# Autodesk Inventor assembly: Z
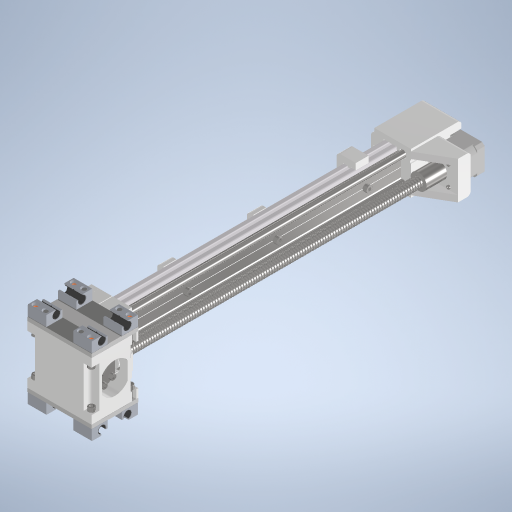
[picture p0: Inventor's stored thumbnail of the model, 512x512]
Saved by Autodesk Inventor 2024 (Build 280153000, 153)
## iProperties
Created: 2022-04-26
Part Number: Z
Document SubType Name: Assembly
Designer: mikoma
Author: mikoma
## Documents named in this file (30)
- D:\@home\mikoma\Dokumenty\DR\CartesianRobotsDigitalTwin\model\Workspaces\Obszar roboczy\assembly_v3\Z\Z.iam
- D:\@home\mikoma\Dokumenty\DR\CartesianRobotsDigitalTwin\model\Workspaces\Obszar roboczy\content\igus\WW_10_40_10_2.ipt
- D:\@home\mikoma\Dokumenty\DR\CartesianRobotsDigitalTwin\model\Workspaces\Obszar roboczy\assembly_v3\Z\ZCarriage.ipt
- D:\@home\mikoma\Dokumenty\DR\CartesianRobotsDigitalTwin\model\Workspaces\Obszar roboczy\content\manipulatorSharedParts\Cartesian1_BallNut.ipt
- D:\@home\mikoma\Dokumenty\DR\CartesianRobotsDigitalTwin\model\Workspaces\Obszar roboczy\content\manipulatorSharedParts\Cartesian2_BallBearing_25x37x7.ipt
- D:\@home\mikoma\Dokumenty\DR\CartesianRobotsDigitalTwin\model\Workspaces\Obszar roboczy\CC\pl-PL\ISO 4762(1)\DIN EN ISO 4762 - M6 x 30.ipt
- D:\@home\mikoma\Dokumenty\DR\CartesianRobotsDigitalTwin\model\Workspaces\Obszar roboczy\assembly_v3\Z\ZCarriageBackHolder.ipt
- D:\@home\mikoma\Dokumenty\DR\CartesianRobotsDigitalTwin\model\Workspaces\Obszar roboczy\assembly_v3\Z\ZCarriageFrontHolder.ipt
- D:\@home\mikoma\Dokumenty\DR\CartesianRobotsDigitalTwin\model\Workspaces\Obszar roboczy\assembly_v3\Z\ZScrewEndCup.ipt
- D:\@home\mikoma\Dokumenty\DR\CartesianRobotsDigitalTwin\model\Workspaces\Obszar roboczy\assembly_v3\Z\WS_10_40_Z.ipt
- D:\@home\mikoma\Dokumenty\DR\CartesianRobotsDigitalTwin\model\Workspaces\Obszar roboczy\content\item\item_0037003_Profile_5_20x20_L=564_1.ipt
- D:\@home\mikoma\Dokumenty\DR\CartesianRobotsDigitalTwin\model\Workspaces\Obszar roboczy\assembly_v3\Z\ZTop.ipt
- D:\@home\mikoma\Dokumenty\DR\CartesianRobotsDigitalTwin\model\Workspaces\Obszar roboczy\content\manipulatorSharedParts\Cartesian1_12_12_Clutch.ipt
- D:\@home\mikoma\Dokumenty\DR\CartesianRobotsDigitalTwin\model\Workspaces\Obszar roboczy\content\manipulatorSharedParts\Cartesian1_TrapezoidalScrew.ipt
- D:\@home\mikoma\Dokumenty\DR\CartesianRobotsDigitalTwin\model\Workspaces\Obszar roboczy\assembly_v3\Z\ZItemMount.ipt
- D:\@home\mikoma\Dokumenty\DR\CartesianRobotsDigitalTwin\model\Workspaces\Obszar roboczy\content\manipulatorSharedParts\stopSw.ipt
- D:\@home\mikoma\Dokumenty\DR\CartesianRobotsDigitalTwin\model\Workspaces\Obszar roboczy\content\manipulatorSharedParts\Connector_female.ipt
- D:\@home\mikoma\Dokumenty\DR\CartesianRobotsDigitalTwin\model\Workspaces\Obszar roboczy\CC\pl-PL\ISO 4762(1)\DIN EN ISO 4762 - M5 x 40.ipt
- D:\@home\mikoma\Dokumenty\DR\CartesianRobotsDigitalTwin\model\Workspaces\Obszar roboczy\CC\pl-PL\ISO 4032(2)\ISO 4032 - M5 - ISO.ipt
- D:\@home\mikoma\Dokumenty\DR\CartesianRobotsDigitalTwin\model\Workspaces\Obszar roboczy\assembly_v3\Z\ZItemMountCable.ipt
- D:\@home\mikoma\Dokumenty\DR\CartesianRobotsDigitalTwin\model\Workspaces\Obszar roboczy\assembly_v3\Z\ZTopCable.ipt
- D:\@home\mikoma\Dokumenty\DR\CartesianRobotsDigitalTwin\model\Workspaces\Obszar roboczy\CC\pl-PL\ISO 4762(2)\ISO 4762 - M4 x 25ISO.ipt
- D:\@home\mikoma\Dokumenty\DR\CartesianRobotsDigitalTwin\model\Workspaces\Obszar roboczy\CC\pl-PL\ISO 4762(1)\DIN EN ISO 4762 - M6 x 25.ipt
- D:\@home\mikoma\Dokumenty\DR\CartesianRobotsDigitalTwin\model\Workspaces\Obszar roboczy\CC\pl-PL\ISO 4762(1)\DIN EN ISO 4762 - M6 x 55.ipt
- D:\@home\mikoma\Dokumenty\DR\CartesianRobotsDigitalTwin\model\Workspaces\Obszar roboczy\CC\pl-PL\ISO 4032(2)\ISO 4032 - M6 - ISO.ipt
- D:\@home\mikoma\Dokumenty\DR\CartesianRobotsDigitalTwin\model\Workspaces\Obszar roboczy\CC\pl-PL\DIN 7984\DIN 7984 - M4 x 14.ipt
- D:\@home\mikoma\Dokumenty\DR\CartesianRobotsDigitalTwin\model\Workspaces\Obszar roboczy\CC\pl-PL\ISO 4762(1)\DIN EN ISO 4762 - M6 x 35.ipt
- D:\@home\mikoma\Dokumenty\DR\CartesianRobotsDigitalTwin\model\Workspaces\Obszar roboczy\CC\pl-PL\DIN 7984\DIN 7984 - M3 x 14.ipt
- D:\@home\mikoma\Dokumenty\DR\CartesianRobotsDigitalTwin\model\Workspaces\Obszar roboczy\content\item\item_0037006_Wpust_przesuwny_5_St_M4_1.ipt
- D:\@home\mikoma\Dokumenty\DR\CartesianRobotsDigitalTwin\model\Workspaces\Obszar roboczy\content\nema17\17HS4401\17HS4401.ipt
## Components (75 placed, 29 different names)
1. WW_10_40_10_2:1 — Zestawiające:14, Zestawiające:15, Zestawiające:18, Zestawiające:19
2. WW_10_40_10_2:2 — Zestawiające:16, Zestawiające:17, Zestawiające:18
3. ZCarriage:1 — Równoległe:2, Zestawiające:13, Równoległe:3, Zestawiające:14, Zestawiające:15, Zestawiające:16, Zestawiające:17, Zestawiające:20, Kątowe:1, Zestawiające:21, Zestawiające:22, Zestawiające:23, Zestawiające:24, Zestawiające:25, Zestawiające:26, Zestawiające:27, Zestawiające:28, Równoległe:4, Równoległe:5, Równoległe:6, Zestawiające:29, Zestawiające:30, Zestawiające:31, Zestawiające:34, Zestawiające:35, Zestawiające:36, Zestawiające:39, Zestawiające:40, Zestawiające:56, Zestawiające:57, Zestawiające:58, Kątowe:3, Zestawiające:62, Zestawiające:80, Zestawiające:81, Zestawiające:82, Zestawiające:83, Zestawiające:84, Zestawiające:85, Zestawiające:86, Zestawiające:87, Zestawiające:88, Zestawiające:89, Zestawiające:90, Zestawiające:91, Kątowe:4, Zestawiające:101, Kątowe:5, Zestawiające:103, Kątowe:6, Zestawiające:105, Kątowe:7, Zestawiające:107, Kątowe:8, Zestawiające:109
4. Cartesian1_BallNut:1 — Zestawiające:20, Kątowe:1, Zestawiające:21, Zestawiające:59, Zestawiające:60, Zestawiające:70, Zestawiające:71, Zestawiające:72, Zestawiające:73, Zestawiające:74, Zestawiające:75, Zestawiające:76, Zestawiające:77, Zestawiające:78, Zestawiające:79
5. Cartesian2_BallBearing_25x37x7:1 — Zestawiające:22, Zestawiające:23
6. ZCarriageBackHolder:1 — Zestawiające:28, Równoległe:4, Równoległe:5, Kątowe:9, Zestawiające:111, Kątowe:10, Zestawiające:113, Kątowe:11, Zestawiające:116, Kątowe:12, Zestawiające:118, Zestawiające:125
7. ZScrewEndCup:1 — Zestawiające:46
8. ZCarriageFrontHolder:1 — Równoległe:6, Zestawiające:29, Zestawiające:30, Zestawiające:31, Zestawiające:32, Zestawiające:33, Równoległe:7, Zestawiające:54, Zestawiające:55, Zestawiające:92, Zestawiające:93, Zestawiające:94, Zestawiające:95, Zestawiające:96, Zestawiające:97, Zestawiające:98, Zestawiające:99
9. WS_10_40_Z:1 — Zestawiające:32, Zestawiające:33, Zestawiające:34, Zestawiające:37, Zestawiające:38, Zestawiające:41, Zestawiające:42, Zestawiające:141, Zestawiające:143, Zestawiające:145
10. item_0037003_Profile_5_20x20_L=564_1:1 — Zestawiające:38, Zestawiające:39, Zestawiające:40, Zestawiające:50, Zestawiające:159, Zestawiające:161, Zestawiające:165, Zestawiające:169
11. item_0037003_Profile_5_20x20_L=564_1:2 — Zestawiające:35, Zestawiające:36, Zestawiające:37, Zestawiające:43, Zestawiające:51, Zestawiające:52, Zestawiające:53, Zestawiające:63, Zestawiające:64, Zestawiające:157, Zestawiające:163, Zestawiające:167, Zestawiające:171
12. ZTop:1 — Zestawiające:41, Zestawiające:42, Zestawiające:43, Zestawiające:49, Zestawiające:65, Zestawiające:66, Zestawiające:67, Zestawiające:148, Zestawiające:149, Zestawiające:150, Zestawiające:151, Zestawiające:152, Zestawiające:153, Zestawiające:154, Zestawiające:155, Mate:174
13. Cartesian1_12_12_Clutch:1 — Zestawiające:47, Zestawiające:48, Zestawiające:49
14. Cartesian1_TrapezoidalScrew:1 — Zestawiające:46, Zestawiające:47, Zestawiające:48
15. ZItemMount:1 — Zestawiające:50, Zestawiające:51, Zestawiające:119, Kątowe:13, Zestawiające:120, Zestawiające:125, Zestawiające:126, Zestawiające:136, Zestawiające:137, Zestawiające:138, Zestawiające:139, Kątowe:16, Kątowe:17
16. ZItemMount:2 — Zestawiające:52, Zestawiające:53, Zestawiające:121, Kątowe:14, Zestawiające:122, Zestawiające:126, Zestawiające:127, Zestawiające:132, Zestawiające:133, Zestawiające:134, Zestawiające:135, Kątowe:18, Kątowe:19
17. stopSw:1 — Równoległe:7, Zestawiające:54, Zestawiające:55
18. Connector_female:1 — Zestawiające:56, Zestawiające:57, Zestawiające:58
19. ZItemMountCable:1 — Zestawiające:63, Zestawiające:64, Zestawiające:123, Kątowe:15, Zestawiające:124, Zestawiające:127, Zestawiające:128, Zestawiające:129, Zestawiające:130, Zestawiające:131, Kątowe:20, Kątowe:21
20. ZTopCable:1 — Zestawiające:65, Zestawiające:66, Zestawiające:67, Zestawiające:146, Zestawiające:147, Kątowe:22, Kątowe:23, Zestawiające:172, Zestawiające:173
21. 17HS4401:1 — Mate:174, Mate:175, Mate:176
22. DIN EN ISO 4762 M6 x 30:2 — Zestawiające:26, Zestawiające:27
23. DIN EN ISO 4762 M6 x 25:1 — Zestawiające:24, Zestawiające:25
24. ISO 4032 M5:1 — Zestawiające:61, Kątowe:3, Zestawiające:62
25. DIN EN ISO 4762 M5 x 40:1 — Zestawiające:59, Zestawiające:60, Zestawiające:61
26. DIN EN ISO 4762 M6 x 30:8 — Zestawiające:90, Zestawiające:91
27. DIN EN ISO 4762 M6 x 30:7 — Zestawiające:88, Zestawiające:89
28. DIN EN ISO 4762 M6 x 30:6 — Zestawiające:86, Zestawiające:87
29. DIN EN ISO 4762 M6 x 30:5 — Zestawiające:84, Zestawiające:85
30. DIN EN ISO 4762 M6 x 30:4 — Zestawiające:82, Zestawiające:83
31. DIN EN ISO 4762 M6 x 25:2 — Zestawiające:80, Zestawiające:81
32. DIN EN ISO 4762 M5 x 40:6 — Zestawiające:74, Zestawiające:77, Zestawiające:104
33. DIN EN ISO 4762 M5 x 40:5 — Zestawiające:73, Zestawiające:78, Zestawiające:106
34. DIN EN ISO 4762 M5 x 40:4 — Zestawiające:72, Zestawiające:79, Zestawiające:108
35. DIN EN ISO 4762 M5 x 40:3 — Zestawiające:71, Zestawiające:75, Zestawiające:102
36. DIN EN ISO 4762 M5 x 40:2 — Zestawiające:70, Zestawiające:76, Zestawiające:100
37. DIN 7984 M3 x 14:4 — Zestawiające:154, Zestawiające:155
38. DIN 7984 M3 x 14:3 — Zestawiające:152, Zestawiające:153, Mate:175
39. DIN 7984 M3 x 14:2 — Zestawiające:150, Zestawiające:151
40. DIN 7984 M3 x 14:1 — Zestawiające:148, Zestawiające:149, Mate:176
41. ISO 4762 M4 x 25:2 — Zestawiające:146, Zestawiające:147, Zestawiające:170
42. DIN EN ISO 4762 M6 x 35:3 — Zestawiające:144, Zestawiające:145
43. DIN EN ISO 4762 M6 x 35:2 — Zestawiające:142, Zestawiające:143
44. DIN EN ISO 4762 M6 x 35:1 — Zestawiające:140, Zestawiające:141
45. DIN 7984 M4 x 14:6 — Zestawiające:138, Zestawiające:139, Zestawiające:156
46. DIN 7984 M4 x 14:5 — Zestawiające:136, Zestawiające:137, Zestawiające:158
47. DIN 7984 M4 x 14:4 — Zestawiające:134, Zestawiające:135, Zestawiające:162
48. DIN 7984 M4 x 14:3 — Zestawiające:132, Zestawiające:133, Zestawiające:160
49. DIN 7984 M4 x 14:2 — Zestawiające:130, Zestawiające:131, Zestawiające:166
50. DIN 7984 M4 x 14:1 — Zestawiające:128, Zestawiające:129, Zestawiające:164
51. ISO 4032 M6:7 — Zestawiające:123, Kątowe:15, Zestawiające:124, Zestawiające:144
52. ISO 4032 M6:6 — Zestawiające:121, Kątowe:14, Zestawiające:122, Zestawiające:142
53. ISO 4032 M6:5 — Zestawiające:119, Kątowe:13, Zestawiające:120, Zestawiające:140
54. ISO 4032 M6:4 — Zestawiające:117, Kątowe:12, Zestawiające:118
55. ISO 4032 M6:3 — Zestawiające:114, Zestawiające:115, Kątowe:11, Zestawiające:116
56. ISO 4032 M6:2 — Zestawiające:112, Kątowe:10, Zestawiające:113
57. ISO 4032 M6:1 — Zestawiające:110, Kątowe:9, Zestawiające:111
58. ISO 4032 M5:6 — Kątowe:8, Zestawiające:108, Zestawiające:109
59. ISO 4032 M5:5 — Kątowe:7, Zestawiające:106, Zestawiające:107
60. ISO 4032 M5:4 — Kątowe:6, Zestawiające:104, Zestawiające:105
61. ISO 4032 M5:3 — Kątowe:5, Zestawiające:102, Zestawiające:103
62. ISO 4032 M5:2 — Zestawiające:100, Kątowe:4, Zestawiające:101
63. DIN EN ISO 4762 M6 x 55:4 — Zestawiające:98, Zestawiające:99, Zestawiające:110
64. DIN EN ISO 4762 M6 x 55:3 — Zestawiające:96, Zestawiające:97, Zestawiające:112
65. DIN EN ISO 4762 M6 x 55:2 — Zestawiające:94, Zestawiające:95, Zestawiające:117
66. DIN EN ISO 4762 M6 x 55:1 — Zestawiające:92, Zestawiające:93, Zestawiające:114, Zestawiające:115
67. item_0037006_Wpust_przesuwny_5_St_M4_1:1 — Zestawiające:156, Kątowe:16, Zestawiające:157
68. item_0037006_Wpust_przesuwny_5_St_M4_1:2 — Zestawiające:158, Kątowe:17, Zestawiające:159
69. item_0037006_Wpust_przesuwny_5_St_M4_1:3 — Zestawiające:160, Kątowe:18, Zestawiające:161
70. item_0037006_Wpust_przesuwny_5_St_M4_1:4 — Zestawiające:162, Kątowe:19, Zestawiające:163
71. item_0037006_Wpust_przesuwny_5_St_M4_1:5 — Zestawiające:164, Kątowe:20, Zestawiające:165
72. item_0037006_Wpust_przesuwny_5_St_M4_1:6 — Zestawiające:166, Kątowe:21, Zestawiające:167
73. item_0037006_Wpust_przesuwny_5_St_M4_1:7 — Kątowe:22, Zestawiające:169
74. item_0037006_Wpust_przesuwny_5_St_M4_1:8 — Zestawiające:170, Kątowe:23, Zestawiające:171
75. ISO 4762 M4 x 25:3 — Zestawiające:172, Zestawiające:173
## Relationships (189: Mate 161, Angle 22, Flush 6)
- [Mate]: Cartesian2_BallBearing_25x37x7:1 ↔ ZScrewEndCup:1
- [Mate]: Cartesian2_BallBearing_25x37x7:1 ↔ ZScrewEndCup:1
- Równoległe:2 [Flush]: ZCarriage:1
- Zestawiające:13 [Mate]: ZCarriage:1
- Równoległe:3 [Flush]: ZCarriage:1
- Zestawiające:14 [Mate]: WW_10_40_10_2:1 ↔ ZCarriage:1
- Zestawiające:15 [Mate]: WW_10_40_10_2:1 ↔ ZCarriage:1
- Zestawiające:16 [Mate]: WW_10_40_10_2:2 ↔ ZCarriage:1
- Zestawiające:17 [Mate]: WW_10_40_10_2:2 ↔ ZCarriage:1
- Zestawiające:18 [Mate] (120 mm): WW_10_40_10_2:1 ↔ WW_10_40_10_2:2
- Zestawiające:19 [Mate] (-67.5 mm): WW_10_40_10_2:1
- Zestawiające:20 [Mate]: ZCarriage:1 ↔ Cartesian1_BallNut:1
- Kątowe:1 [Angle] (0 deg): ZCarriage:1 ↔ Cartesian1_BallNut:1
- Zestawiające:21 [Mate]: ZCarriage:1 ↔ Cartesian1_BallNut:1
- Zestawiające:22 [Mate]: ZCarriage:1 ↔ Cartesian2_BallBearing_25x37x7:1
- Zestawiające:23 [Mate]: ZCarriage:1 ↔ Cartesian2_BallBearing_25x37x7:1
- Zestawiające:24 [Mate]: ZCarriage:1 ↔ DIN EN ISO 4762 M6 x 25:1
- Zestawiające:25 [Mate]: ZCarriage:1 ↔ DIN EN ISO 4762 M6 x 25:1
- Zestawiające:26 [Mate]: ZCarriage:1 ↔ DIN EN ISO 4762 M6 x 30:2
- Zestawiające:27 [Mate]: ZCarriage:1 ↔ DIN EN ISO 4762 M6 x 30:2
- Zestawiające:28 [Mate]: ZCarriage:1 ↔ ZCarriageBackHolder:1
- Równoległe:4 [Flush]: ZCarriage:1 ↔ ZCarriageBackHolder:1
- Równoległe:5 [Flush]: ZCarriage:1 ↔ ZCarriageBackHolder:1
- Równoległe:6 [Flush]: ZCarriage:1 ↔ ZCarriageFrontHolder:1
- Zestawiające:29 [Mate]: ZCarriage:1 ↔ ZCarriageFrontHolder:1
- Zestawiające:30 [Mate]: ZCarriage:1 ↔ ZCarriageFrontHolder:1
- Zestawiające:31 [Mate]: ZCarriage:1 ↔ ZCarriageFrontHolder:1
- Zestawiające:32 [Mate]: ZCarriageFrontHolder:1 ↔ WS_10_40_Z:1
- Zestawiające:33 [Mate]: ZCarriageFrontHolder:1 ↔ WS_10_40_Z:1
- Zestawiające:34 [Mate]: ZCarriage:1 ↔ WS_10_40_Z:1
- Zestawiające:35 [Mate]: ZCarriage:1 ↔ item_0037003_Profile_5_20x20_L=564_1:2
- Zestawiające:36 [Mate]: ZCarriage:1 ↔ item_0037003_Profile_5_20x20_L=564_1:2
- Zestawiające:37 [Mate]: WS_10_40_Z:1 ↔ item_0037003_Profile_5_20x20_L=564_1:2
- Zestawiające:38 [Mate]: WS_10_40_Z:1 ↔ item_0037003_Profile_5_20x20_L=564_1:1
- Zestawiające:39 [Mate]: ZCarriage:1 ↔ item_0037003_Profile_5_20x20_L=564_1:1
- Zestawiające:40 [Mate]: ZCarriage:1 ↔ item_0037003_Profile_5_20x20_L=564_1:1
- Zestawiające:41 [Mate]: WS_10_40_Z:1 ↔ ZTop:1
- Zestawiające:42 [Mate]: WS_10_40_Z:1 ↔ ZTop:1
- Zestawiające:43 [Mate]: item_0037003_Profile_5_20x20_L=564_1:2 ↔ ZTop:1
- Zestawiające:46 [Mate]: ZScrewEndCup:1 ↔ Cartesian1_TrapezoidalScrew:1
- Zestawiające:47 [Mate]: Cartesian1_12_12_Clutch:1 ↔ Cartesian1_TrapezoidalScrew:1
- Zestawiające:48 [Mate]: Cartesian1_12_12_Clutch:1 ↔ Cartesian1_TrapezoidalScrew:1
- Zestawiające:49 [Mate]: ZTop:1 ↔ Cartesian1_12_12_Clutch:1
- Zestawiające:50 [Mate]: item_0037003_Profile_5_20x20_L=564_1:1 ↔ ZItemMount:1
- Zestawiające:51 [Mate]: item_0037003_Profile_5_20x20_L=564_1:2 ↔ ZItemMount:1
- Zestawiające:52 [Mate]: item_0037003_Profile_5_20x20_L=564_1:2 ↔ ZItemMount:2
- Zestawiające:53 [Mate]: item_0037003_Profile_5_20x20_L=564_1:2 ↔ ZItemMount:2
- Równoległe:7 [Flush] (-1 mm): ZCarriageFrontHolder:1 ↔ stopSw:1
- Zestawiające:54 [Mate]: ZCarriageFrontHolder:1 ↔ stopSw:1
- Zestawiające:55 [Mate]: ZCarriageFrontHolder:1 ↔ stopSw:1
- Zestawiające:56 [Mate]: ZCarriage:1 ↔ Connector_female:1
- Zestawiające:57 [Mate]: ZCarriage:1 ↔ Connector_female:1
- Zestawiające:58 [Mate]: ZCarriage:1 ↔ Connector_female:1
- Zestawiające:59 [Mate]: Cartesian1_BallNut:1 ↔ DIN EN ISO 4762 M5 x 40:1
- Zestawiające:60 [Mate]: Cartesian1_BallNut:1 ↔ DIN EN ISO 4762 M5 x 40:1
- Zestawiające:61 [Mate]: ISO 4032 M5:1 ↔ DIN EN ISO 4762 M5 x 40:1
- Kątowe:3 [Angle] (0 deg): ZCarriage:1 ↔ ISO 4032 M5:1
- Zestawiające:62 [Mate]: ZCarriage:1 ↔ ISO 4032 M5:1
- Zestawiające:63 [Mate]: item_0037003_Profile_5_20x20_L=564_1:2 ↔ ZItemMountCable:1
- Zestawiające:64 [Mate]: item_0037003_Profile_5_20x20_L=564_1:2 ↔ ZItemMountCable:1
- Zestawiające:65 [Mate]: ZTop:1 ↔ ZTopCable:1
- Zestawiające:66 [Mate]: ZTop:1 ↔ ZTopCable:1
- Zestawiające:67 [Mate]: ZTop:1 ↔ ZTopCable:1
- Zestawiające:70 [Mate]: Cartesian1_BallNut:1 ↔ DIN EN ISO 4762 M5 x 40:2
- Zestawiające:71 [Mate]: Cartesian1_BallNut:1 ↔ DIN EN ISO 4762 M5 x 40:3
- Zestawiające:72 [Mate]: Cartesian1_BallNut:1 ↔ DIN EN ISO 4762 M5 x 40:4
- Zestawiające:73 [Mate]: Cartesian1_BallNut:1 ↔ DIN EN ISO 4762 M5 x 40:5
- Zestawiające:74 [Mate]: Cartesian1_BallNut:1 ↔ DIN EN ISO 4762 M5 x 40:6
- Zestawiające:75 [Mate]: Cartesian1_BallNut:1 ↔ DIN EN ISO 4762 M5 x 40:3
- Zestawiające:76 [Mate]: Cartesian1_BallNut:1 ↔ DIN EN ISO 4762 M5 x 40:2
- Zestawiające:77 [Mate]: Cartesian1_BallNut:1 ↔ DIN EN ISO 4762 M5 x 40:6
- Zestawiające:78 [Mate]: Cartesian1_BallNut:1 ↔ DIN EN ISO 4762 M5 x 40:5
- Zestawiające:79 [Mate]: Cartesian1_BallNut:1 ↔ DIN EN ISO 4762 M5 x 40:4
- Zestawiające:80 [Mate]: ZCarriage:1 ↔ DIN EN ISO 4762 M6 x 25:2
- Zestawiające:81 [Mate]: ZCarriage:1 ↔ DIN EN ISO 4762 M6 x 25:2
- Zestawiające:82 [Mate]: ZCarriage:1 ↔ DIN EN ISO 4762 M6 x 30:4
- Zestawiające:83 [Mate]: ZCarriage:1 ↔ DIN EN ISO 4762 M6 x 30:4
- Zestawiające:84 [Mate]: ZCarriage:1 ↔ DIN EN ISO 4762 M6 x 30:5
- Zestawiające:85 [Mate]: ZCarriage:1 ↔ DIN EN ISO 4762 M6 x 30:5
- Zestawiające:86 [Mate]: ZCarriage:1 ↔ DIN EN ISO 4762 M6 x 30:6
- Zestawiające:87 [Mate]: ZCarriage:1 ↔ DIN EN ISO 4762 M6 x 30:6
- Zestawiające:88 [Mate]: ZCarriage:1 ↔ DIN EN ISO 4762 M6 x 30:7
- Zestawiające:89 [Mate]: ZCarriage:1 ↔ DIN EN ISO 4762 M6 x 30:7
- Zestawiające:90 [Mate]: ZCarriage:1 ↔ DIN EN ISO 4762 M6 x 30:8
- Zestawiające:91 [Mate]: ZCarriage:1 ↔ DIN EN ISO 4762 M6 x 30:8
- Zestawiające:92 [Mate]: ZCarriageFrontHolder:1 ↔ DIN EN ISO 4762 M6 x 55:1
- Zestawiające:93 [Mate]: ZCarriageFrontHolder:1 ↔ DIN EN ISO 4762 M6 x 55:1
- Zestawiające:94 [Mate]: ZCarriageFrontHolder:1 ↔ DIN EN ISO 4762 M6 x 55:2
- Zestawiające:95 [Mate]: ZCarriageFrontHolder:1 ↔ DIN EN ISO 4762 M6 x 55:2
- Zestawiające:96 [Mate]: ZCarriageFrontHolder:1 ↔ DIN EN ISO 4762 M6 x 55:3
- Zestawiające:97 [Mate]: ZCarriageFrontHolder:1 ↔ DIN EN ISO 4762 M6 x 55:3
- Zestawiające:98 [Mate]: ZCarriageFrontHolder:1 ↔ DIN EN ISO 4762 M6 x 55:4
- Zestawiające:99 [Mate]: ZCarriageFrontHolder:1 ↔ DIN EN ISO 4762 M6 x 55:4
- Zestawiające:100 [Mate]: DIN EN ISO 4762 M5 x 40:2 ↔ ISO 4032 M5:2
- Kątowe:4 [Angle] (0 deg): ZCarriage:1 ↔ ISO 4032 M5:2
- Zestawiające:101 [Mate]: ZCarriage:1 ↔ ISO 4032 M5:2
- Kątowe:5 [Angle] (0 deg): ZCarriage:1 ↔ ISO 4032 M5:3
- Zestawiające:102 [Mate]: DIN EN ISO 4762 M5 x 40:3 ↔ ISO 4032 M5:3
- Zestawiające:103 [Mate]: ZCarriage:1 ↔ ISO 4032 M5:3
- Kątowe:6 [Angle] (0 deg): ZCarriage:1 ↔ ISO 4032 M5:4
- Zestawiające:104 [Mate]: DIN EN ISO 4762 M5 x 40:6 ↔ ISO 4032 M5:4
- Zestawiające:105 [Mate]: ZCarriage:1 ↔ ISO 4032 M5:4
- Kątowe:7 [Angle] (0 deg): ZCarriage:1 ↔ ISO 4032 M5:5
- Zestawiające:106 [Mate]: DIN EN ISO 4762 M5 x 40:5 ↔ ISO 4032 M5:5
- Zestawiające:107 [Mate]: ZCarriage:1 ↔ ISO 4032 M5:5
- Kątowe:8 [Angle] (0 deg): ZCarriage:1 ↔ ISO 4032 M5:6
- Zestawiające:108 [Mate]: DIN EN ISO 4762 M5 x 40:4 ↔ ISO 4032 M5:6
- Zestawiające:109 [Mate]: ZCarriage:1 ↔ ISO 4032 M5:6
- Zestawiające:110 [Mate]: ISO 4032 M6:1 ↔ DIN EN ISO 4762 M6 x 55:4
- Kątowe:9 [Angle] (0 deg): ZCarriageBackHolder:1 ↔ ISO 4032 M6:1
- Zestawiające:111 [Mate]: ZCarriageBackHolder:1 ↔ ISO 4032 M6:1
- Zestawiające:112 [Mate]: ISO 4032 M6:2 ↔ DIN EN ISO 4762 M6 x 55:3
- Kątowe:10 [Angle] (0 deg): ZCarriageBackHolder:1 ↔ ISO 4032 M6:2
- Zestawiające:113 [Mate]: ZCarriageBackHolder:1 ↔ ISO 4032 M6:2
- Zestawiające:114 [Mate]: ISO 4032 M6:3 ↔ DIN EN ISO 4762 M6 x 55:1
- Zestawiające:115 [Mate]: ISO 4032 M6:3 ↔ DIN EN ISO 4762 M6 x 55:1
- Kątowe:11 [Angle] (0 deg): ZCarriageBackHolder:1 ↔ ISO 4032 M6:3
- Zestawiające:116 [Mate]: ZCarriageBackHolder:1 ↔ ISO 4032 M6:3
- Zestawiające:117 [Mate]: ISO 4032 M6:4 ↔ DIN EN ISO 4762 M6 x 55:2
- Kątowe:12 [Angle] (0 deg): ZCarriageBackHolder:1 ↔ ISO 4032 M6:4
- Zestawiające:118 [Mate]: ZCarriageBackHolder:1 ↔ ISO 4032 M6:4
- Zestawiające:119 [Mate]: ZItemMount:1 ↔ ISO 4032 M6:5
- Kątowe:13 [Angle] (0 deg): ZItemMount:1 ↔ ISO 4032 M6:5
- Zestawiające:120 [Mate]: ZItemMount:1 ↔ ISO 4032 M6:5
- Zestawiające:121 [Mate]: ZItemMount:2 ↔ ISO 4032 M6:6
- Kątowe:14 [Angle] (0 deg): ZItemMount:2 ↔ ISO 4032 M6:6
- Zestawiające:122 [Mate]: ZItemMount:2 ↔ ISO 4032 M6:6
- Zestawiające:123 [Mate]: ZItemMountCable:1 ↔ ISO 4032 M6:7
- Kątowe:15 [Angle] (0 deg): ZItemMountCable:1 ↔ ISO 4032 M6:7
- Zestawiające:124 [Mate]: ZItemMountCable:1 ↔ ISO 4032 M6:7
- Zestawiające:125 [Mate] (100 mm): ZCarriageBackHolder:1 ↔ ZItemMount:1
- Zestawiające:126 [Mate] (120 mm): ZItemMount:1 ↔ ZItemMount:2
- Zestawiające:127 [Mate] (120 mm): ZItemMount:2 ↔ ZItemMountCable:1
- Zestawiające:128 [Mate]: ZItemMountCable:1 ↔ DIN 7984 M4 x 14:1
- Zestawiające:129 [Mate]: ZItemMountCable:1 ↔ DIN 7984 M4 x 14:1
- Zestawiające:130 [Mate]: ZItemMountCable:1 ↔ DIN 7984 M4 x 14:2
- Zestawiające:131 [Mate]: ZItemMountCable:1 ↔ DIN 7984 M4 x 14:2
- Zestawiające:132 [Mate]: ZItemMount:2 ↔ DIN 7984 M4 x 14:3
- Zestawiające:133 [Mate]: ZItemMount:2 ↔ DIN 7984 M4 x 14:3
- Zestawiające:134 [Mate]: ZItemMount:2 ↔ DIN 7984 M4 x 14:4
- Zestawiające:135 [Mate]: ZItemMount:2 ↔ DIN 7984 M4 x 14:4
- Zestawiające:136 [Mate]: ZItemMount:1 ↔ DIN 7984 M4 x 14:5
- Zestawiające:137 [Mate]: ZItemMount:1 ↔ DIN 7984 M4 x 14:5
- Zestawiające:138 [Mate]: ZItemMount:1 ↔ DIN 7984 M4 x 14:6
- Zestawiające:139 [Mate]: ZItemMount:1 ↔ DIN 7984 M4 x 14:6
- Zestawiające:140 [Mate]: DIN EN ISO 4762 M6 x 35:1 ↔ ISO 4032 M6:5
- Zestawiające:141 [Mate]: WS_10_40_Z:1 ↔ DIN EN ISO 4762 M6 x 35:1
- Zestawiające:142 [Mate]: DIN EN ISO 4762 M6 x 35:2 ↔ ISO 4032 M6:6
- Zestawiające:143 [Mate]: WS_10_40_Z:1 ↔ DIN EN ISO 4762 M6 x 35:2
- Zestawiające:144 [Mate]: DIN EN ISO 4762 M6 x 35:3 ↔ ISO 4032 M6:7
- Zestawiające:145 [Mate]: WS_10_40_Z:1 ↔ DIN EN ISO 4762 M6 x 35:3
- Zestawiające:146 [Mate]: ZTopCable:1 ↔ ISO 4762 M4 x 25:2
- Zestawiające:147 [Mate]: ZTopCable:1 ↔ ISO 4762 M4 x 25:2
- Zestawiające:148 [Mate]: ZTop:1 ↔ DIN 7984 M3 x 14:1
- Zestawiające:149 [Mate]: ZTop:1 ↔ DIN 7984 M3 x 14:1
- Zestawiające:150 [Mate]: ZTop:1 ↔ DIN 7984 M3 x 14:2
- Zestawiające:151 [Mate]: ZTop:1 ↔ DIN 7984 M3 x 14:2
- Zestawiające:152 [Mate]: ZTop:1 ↔ DIN 7984 M3 x 14:3
- Zestawiające:153 [Mate]: ZTop:1 ↔ DIN 7984 M3 x 14:3
- Zestawiające:154 [Mate]: ZTop:1 ↔ DIN 7984 M3 x 14:4
- Zestawiające:155 [Mate]: ZTop:1 ↔ DIN 7984 M3 x 14:4
- Zestawiające:156 [Mate]: DIN 7984 M4 x 14:6 ↔ item_0037006_Wpust_przesuwny_5_St_M4_1:1
- Kątowe:16 [Angle] (0 deg): ZItemMount:1 ↔ item_0037006_Wpust_przesuwny_5_St_M4_1:1
- Zestawiające:157 [Mate]: item_0037003_Profile_5_20x20_L=564_1:2 ↔ item_0037006_Wpust_przesuwny_5_St_M4_1:1
- Zestawiające:158 [Mate]: DIN 7984 M4 x 14:5 ↔ item_0037006_Wpust_przesuwny_5_St_M4_1:2
- Kątowe:17 [Angle] (0 deg): ZItemMount:1 ↔ item_0037006_Wpust_przesuwny_5_St_M4_1:2
- Zestawiające:159 [Mate]: item_0037003_Profile_5_20x20_L=564_1:1 ↔ item_0037006_Wpust_przesuwny_5_St_M4_1:2
- Zestawiające:160 [Mate]: DIN 7984 M4 x 14:3 ↔ item_0037006_Wpust_przesuwny_5_St_M4_1:3
- Kątowe:18 [Angle] (0 deg): ZItemMount:2 ↔ item_0037006_Wpust_przesuwny_5_St_M4_1:3
- Zestawiające:161 [Mate]: item_0037003_Profile_5_20x20_L=564_1:1 ↔ item_0037006_Wpust_przesuwny_5_St_M4_1:3
- Zestawiające:162 [Mate]: DIN 7984 M4 x 14:4 ↔ item_0037006_Wpust_przesuwny_5_St_M4_1:4
- Kątowe:19 [Angle] (0 deg): ZItemMount:2 ↔ item_0037006_Wpust_przesuwny_5_St_M4_1:4
- Zestawiające:163 [Mate]: item_0037003_Profile_5_20x20_L=564_1:2 ↔ item_0037006_Wpust_przesuwny_5_St_M4_1:4
- Zestawiające:164 [Mate]: DIN 7984 M4 x 14:1 ↔ item_0037006_Wpust_przesuwny_5_St_M4_1:5
- Kątowe:20 [Angle] (0 deg): ZItemMountCable:1 ↔ item_0037006_Wpust_przesuwny_5_St_M4_1:5
- Zestawiające:165 [Mate]: item_0037003_Profile_5_20x20_L=564_1:1 ↔ item_0037006_Wpust_przesuwny_5_St_M4_1:5
- Zestawiające:166 [Mate]: DIN 7984 M4 x 14:2 ↔ item_0037006_Wpust_przesuwny_5_St_M4_1:6
- Kątowe:21 [Angle] (0 deg): ZItemMountCable:1 ↔ item_0037006_Wpust_przesuwny_5_St_M4_1:6
- Zestawiające:167 [Mate]: item_0037003_Profile_5_20x20_L=564_1:2 ↔ item_0037006_Wpust_przesuwny_5_St_M4_1:6
- Kątowe:22 [Angle] (0 deg): ZTopCable:1 ↔ item_0037006_Wpust_przesuwny_5_St_M4_1:7
- Zestawiające:169 [Mate]: item_0037003_Profile_5_20x20_L=564_1:1 ↔ item_0037006_Wpust_przesuwny_5_St_M4_1:7
- Zestawiające:170 [Mate]: ISO 4762 M4 x 25:2 ↔ item_0037006_Wpust_przesuwny_5_St_M4_1:8
- Kątowe:23 [Angle] (0 deg): ZTopCable:1 ↔ item_0037006_Wpust_przesuwny_5_St_M4_1:8
- Zestawiające:171 [Mate]: item_0037003_Profile_5_20x20_L=564_1:2 ↔ item_0037006_Wpust_przesuwny_5_St_M4_1:8
- Zestawiające:172 [Mate]: ZTopCable:1 ↔ ISO 4762 M4 x 25:3
- Zestawiające:173 [Mate]: ZTopCable:1 ↔ ISO 4762 M4 x 25:3
- Mate:174: ZTop:1 ↔ 17HS4401:1
- Mate:175: 17HS4401:1 ↔ DIN 7984 M3 x 14:3
- Mate:176: 17HS4401:1 ↔ DIN 7984 M3 x 14:1
